# Autodesk Inventor assembly: asmTemp
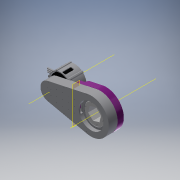
[picture p0: Inventor's stored thumbnail of the model, 180x180]
Saved by Autodesk Inventor 2018 (Build 220112000, 112)
## iProperties
Created: 2019-11-13
Part Number: asmTemp
Document SubType Name: Assembly
Designer: Bunny320
Author: Bunny320
## Documents named in this file (10)
- C:\Users\Bunny320\Desktop\sechs\4-CAD\asmTemp.iam
- C:\Users\Bunny320\Desktop\sechs\4-CAD\101-bottom.ipt
- C:\Users\Bunny320\Desktop\sechs\4-CAD\generated\J1_belt.iam
- C:\Users\Bunny320\Desktop\sechs\4-CAD\standardParts\61814-2RS1\61814-2RS1.iam
- C:\Users\Bunny320\Desktop\sechs\4-CAD\AS5047.ipt
- C:\Users\Bunny320\Desktop\sechs\4-CAD\magnet-6x2.5.ipt
- C:\Users\Bunny320\Desktop\sechs\4-CAD\102-top-motor.ipt
- C:\Users\Bunny320\Desktop\sechs\4-CAD\103-top-output.ipt
- C:\Users\Bunny320\Desktop\sechs\4-CAD\standardParts\SUNNYSKY-X6215S-kv170\X6215S.ipt
- C:\Users\Bunny320\Desktop\sechs\4-CAD\104-motor-case-new.ipt
## Components (10 placed, 9 different names)
1. 101-bottom:1 — Flush:1, Flush:2, Flush:3, Mate:5, Mate:15, Mate:16, Flush:4, Mate:17, Mate:18
2. J1_belt:1 [sub-assembly] — Mate:1, Mate:2, Mate:3, Mate:6, Mate:7, Mate:8, Mate:9, Mate:10, Mate:20, Mate:26
3. 61814-2RS1:1 [sub-assembly] — Mate:2, Mate:8
4. 61814-2RS1:2 [sub-assembly] — Mate:3, Mate:5, Mate:7
5. AS5047:1 — Mate:21, Mate:22, Mate:23
6. magnet-6x2.5:1 — Mate:9, Mate:10
7. 102-top-motor:1 — Mate:15, Mate:16, Flush:4, Mate:19
8. 103-top-output:1 — Mate:17, Mate:18
9. X6215S:1 — Mate:19, Mate:24, Mate:25, Mate:26
10. 104-motor-case-new:1 — Mate:20, Mate:21, Mate:22, Mate:23, Mate:24, Mate:25
## Relationships (25: Mate 21, Flush 4)
- Flush:1: 101-bottom:1
- Flush:2: 101-bottom:1
- Flush:3: 101-bottom:1
- Mate:1: J1_belt:1
- Mate:2: J1_belt:1 ↔ 61814-2RS1:1
- Mate:3: J1_belt:1 ↔ 61814-2RS1:2
- Mate:5: 101-bottom:1 ↔ 61814-2RS1:2
- Mate:6: J1_belt:1
- Mate:7: J1_belt:1 ↔ 61814-2RS1:2
- Mate:8: J1_belt:1 ↔ 61814-2RS1:1
- Mate:9: J1_belt:1 ↔ magnet-6x2.5:1
- Mate:10: J1_belt:1 ↔ magnet-6x2.5:1
- Mate:15: 101-bottom:1 ↔ 102-top-motor:1
- Mate:16: 101-bottom:1 ↔ 102-top-motor:1
- Flush:4: 101-bottom:1 ↔ 102-top-motor:1
- Mate:17: 101-bottom:1 ↔ 103-top-output:1
- Mate:18: 101-bottom:1 ↔ 103-top-output:1
- Mate:19: 102-top-motor:1 ↔ X6215S:1
- Mate:20: J1_belt:1 ↔ 104-motor-case-new:1
- Mate:21: AS5047:1 ↔ 104-motor-case-new:1
- Mate:22: AS5047:1 ↔ 104-motor-case-new:1
- Mate:23: AS5047:1 ↔ 104-motor-case-new:1
- Mate:24: X6215S:1 ↔ 104-motor-case-new:1
- Mate:25: X6215S:1 ↔ 104-motor-case-new:1
- Mate:26: J1_belt:1 ↔ X6215S:1
